# Autodesk Inventor assembly: DIFF_HOUSING_FINAL_ASM
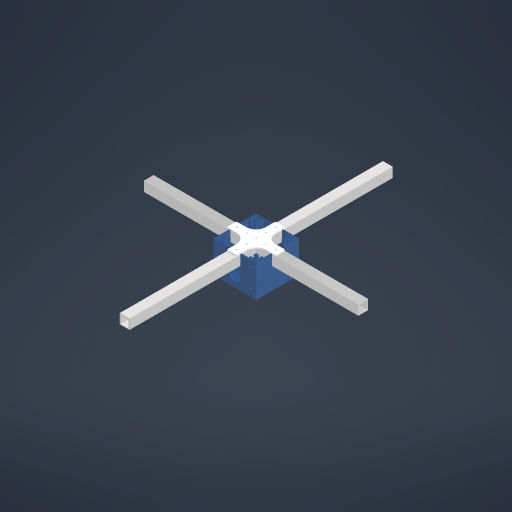
[picture p0: Inventor's stored thumbnail of the model, 512x512]
Saved by Autodesk Inventor 2024 (Build 280153000, 153)
## iProperties
Created: 2023-11-30
Part Number: DIFF_HOUSING_FINAL_ASM
Document SubType Name: Assembly
Designer: bugme
Author: bugme
## Documents named in this file (8)
- C:\Users\bugme\OneDrive - The Pennsylvania State University\Desktop\BRCRP\DIFF_HOUSING_FINAL_ASM.iam
- C:\Users\bugme\OneDrive - The Pennsylvania State University\Desktop\BRCRP\DIFF_HOUSING_WIP.ipt
- C:\Users\bugme\OneDrive - The Pennsylvania State University\Desktop\BRCRP\CH-1-01-20x20 Channel.ipt
- C:\Users\bugme\OneDrive - The Pennsylvania State University\Desktop\BRCRP\DIFF_HOUSING_TOP.ipt
- C:\Users\bugme\OneDrive - The Pennsylvania State University\Desktop\BRCRP\CH-1-01-20x20 Channel\CH-1-01-20x20 Channel-3.13.ipt
- C:\Users\bugme\OneDrive - The Pennsylvania State University\Documents\GitHub\BehrendURCMechanical\CAD\Chassis V3\Body\am-4159 1IN Quad Gusset.ipt
- C:\Users\bugme\OneDrive - The Pennsylvania State University\Documents\GitHub\BehrendURCMechanical\CAD\Chassis V3\Body\44.92cmTube.ipt
- C:\Users\bugme\OneDrive - The Pennsylvania State University\Documents\GitHub\BehrendURCMechanical\CAD\Chassis V3\Body\54.92Shaft.ipt
## Components (11 placed, 6 different names)
1. DIFF_HOUSING_WIP:1 — Mate:1, Mate:2, Flush:1, Mate:3, Mate:4, Flush:2, Mate:5, Mate:6, Flush:3, Mate:7, Mate:8, Flush:4, Flush:5, Flush:6, Flush:7, Flush:8, Mate:14, Mate:16, Mate:19, Mate:22
2. CH-1-01-20x20 Channel-3.13:1 — Mate:1, Mate:2, Flush:1, Mate:10
3. CH-1-01-20x20 Channel-3.13:2 — Mate:3, Mate:4, Flush:2, Mate:9
4. CH-1-01-20x20 Channel-3.13:3 — Mate:5, Mate:6, Flush:3
5. CH-1-01-20x20 Channel-3.13:4 — Mate:7, Mate:8, Flush:4
6. DIFF_HOUSING_TOP:1 — Mate:9, Flush:5, Flush:6
7. DIFF_HOUSING_TOP:2 — Mate:10, Flush:7, Flush:8
8. am-4159 1IN Quad Gusset:1 — Mate:11, Mate:12, Mate:13, Mate:14, Mate:15, Mate:18, Mate:20
9. 44.92cmTube:1 — Mate:15, Mate:16, Mate:17, Mate:21, Mate:23
10. 54.92Shaft:1 — Mate:17, Mate:18, Mate:19
11. 54.92Shaft:2 — Mate:20, Mate:21, Mate:22
## Relationships (31: Mate 23, Flush 8)
- Mate:1: DIFF_HOUSING_WIP:1 ↔ CH-1-01-20x20 Channel-3.13:1
- Mate:2: DIFF_HOUSING_WIP:1 ↔ CH-1-01-20x20 Channel-3.13:1
- Flush:1: DIFF_HOUSING_WIP:1 ↔ CH-1-01-20x20 Channel-3.13:1
- Mate:3: DIFF_HOUSING_WIP:1 ↔ CH-1-01-20x20 Channel-3.13:2
- Mate:4: DIFF_HOUSING_WIP:1 ↔ CH-1-01-20x20 Channel-3.13:2
- Flush:2: DIFF_HOUSING_WIP:1 ↔ CH-1-01-20x20 Channel-3.13:2
- Mate:5: DIFF_HOUSING_WIP:1 ↔ CH-1-01-20x20 Channel-3.13:3
- Mate:6: DIFF_HOUSING_WIP:1 ↔ CH-1-01-20x20 Channel-3.13:3
- Flush:3: DIFF_HOUSING_WIP:1 ↔ CH-1-01-20x20 Channel-3.13:3
- Mate:7: DIFF_HOUSING_WIP:1 ↔ CH-1-01-20x20 Channel-3.13:4
- Mate:8: DIFF_HOUSING_WIP:1 ↔ CH-1-01-20x20 Channel-3.13:4
- Flush:4: DIFF_HOUSING_WIP:1 ↔ CH-1-01-20x20 Channel-3.13:4
- Mate:9: CH-1-01-20x20 Channel-3.13:2 ↔ DIFF_HOUSING_TOP:1
- Flush:5: DIFF_HOUSING_WIP:1 ↔ DIFF_HOUSING_TOP:1
- Flush:6: DIFF_HOUSING_WIP:1 ↔ DIFF_HOUSING_TOP:1
- Mate:10: CH-1-01-20x20 Channel-3.13:1 ↔ DIFF_HOUSING_TOP:2
- Flush:7: DIFF_HOUSING_WIP:1 ↔ DIFF_HOUSING_TOP:2
- Flush:8: DIFF_HOUSING_WIP:1 ↔ DIFF_HOUSING_TOP:2
- Mate:11: am-4159 1IN Quad Gusset:1
- Mate:12: am-4159 1IN Quad Gusset:1
- Mate:13: am-4159 1IN Quad Gusset:1
- Mate:14: DIFF_HOUSING_WIP:1 ↔ am-4159 1IN Quad Gusset:1
- Mate:15: am-4159 1IN Quad Gusset:1 ↔ 44.92cmTube:1
- Mate:16 (1.651 mm): DIFF_HOUSING_WIP:1 ↔ 44.92cmTube:1
- Mate:17: 44.92cmTube:1 ↔ 54.92Shaft:1
- Mate:18: am-4159 1IN Quad Gusset:1 ↔ 54.92Shaft:1
- Mate:19 (1.651 mm): DIFF_HOUSING_WIP:1 ↔ 54.92Shaft:1
- Mate:20: am-4159 1IN Quad Gusset:1 ↔ 54.92Shaft:2
- Mate:21: 44.92cmTube:1 ↔ 54.92Shaft:2
- Mate:22 (1.651 mm): DIFF_HOUSING_WIP:1 ↔ 54.92Shaft:2
- Mate:23 (279.4 mm): 44.92cmTube:1
